# Autodesk Inventor assembly: Pass_Hang_subass
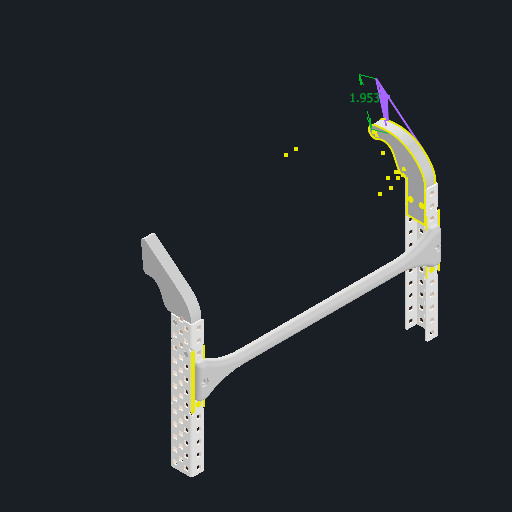
[picture p0: Inventor's stored thumbnail of the model, 512x512]
Saved by Autodesk Inventor 2025.1 (Build 291241000, 241)
## iProperties
Created: 2025-01-10
Part Number: Pass_Hang_subass
Document SubType Name: Assembly
Designer: Juanl
Author: Juanl
## Documents named in this file (5)
- C:\Users\Juanl\Documents\GitHub\ATUM-V5RC-High-Stakes-CAD\Robot\Subassemblies\Pass_Hang_subass.iam
- C:\Users\Juanl\Documents\GitHub\ATUM-V5RC-High-Stakes-CAD\Protobot\Pass_Hang_Hook.ipt
- C:\Users\Juanl\Documents\GitHub\ATUM-V5RC-High-Stakes-CAD\Protobot\Pass_Hang_Hook_MIR.ipt
- C:\Users\Juanl\Documents\GitHub\ATUM-V5RC-High-Stakes-CAD\VEX-CAD-Inventor\Structure\C Channel\Aluminum 1x2x1\Alu C 1x2x1x12.ipt
- C:\Users\Juanl\Documents\GitHub\ATUM-V5RC-High-Stakes-CAD\Additional Parts\Hang_Brace.ipt
## Components (5 placed, 4 different names)
1. Pass_Hang_Hook:1 — Mate:3, Mate:4, Mate:5
2. Pass_Hang_Hook_MIR:1 — Mate:1, Mate:2, Mate:5
3. Alu C 1x2x1x12:2 — Flush:1, Mate:3, Mate:4, Mate:6, Mate:8, Mate:9
4. Alu C 1x2x1x12:1 — Flush:1, Mate:1, Mate:2, Mate:6, Mate:7
5. Hang_Brace:1 — Mate:7, Mate:8, Mate:9
## Relationships (10: Mate 9, Flush 1)
- Flush:1: Alu C 1x2x1x12:2 ↔ Alu C 1x2x1x12:1
- Mate:1: Pass_Hang_Hook_MIR:1 ↔ Alu C 1x2x1x12:1
- Mate:2: Pass_Hang_Hook_MIR:1 ↔ Alu C 1x2x1x12:1
- Mate:3: Pass_Hang_Hook:1 ↔ Alu C 1x2x1x12:2
- Mate:4: Pass_Hang_Hook:1 ↔ Alu C 1x2x1x12:2
- Mate:5: Pass_Hang_Hook:1 ↔ Pass_Hang_Hook_MIR:1
- Mate:6 (282.5496 mm): Alu C 1x2x1x12:2 ↔ Alu C 1x2x1x12:1
- Mate:7: Alu C 1x2x1x12:1 ↔ Hang_Brace:1
- Mate:8: Alu C 1x2x1x12:2 ↔ Hang_Brace:1
- Mate:9: Alu C 1x2x1x12:2 ↔ Hang_Brace:1
